# Autodesk Inventor assembly: Assembly
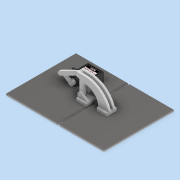
[picture p0: Inventor's stored thumbnail of the model, 180x180]
Saved by Autodesk Inventor 2020 (Build 240168000, 168)
## iProperties
Created: 2020-07-26
Part Number: Assembly
Document SubType Name: Assembly
Designer: Aarya
Author: Aarya
## Documents named in this file (10)
- C:\Users\Aarya\Downloads\R2D2_-_Servo_Driven_Hinge_Design\r2d2\Assembly.iam
- C:\Users\Aarya\Downloads\R2D2_-_Servo_Driven_Hinge_Design\r2d2\plate.ipt
- C:\Users\Aarya\Downloads\R2D2_-_Servo_Driven_Hinge_Design\r2d2\Hinge_Base.ipt
- C:\Users\Aarya\Downloads\R2D2_-_Servo_Driven_Hinge_Design\r2d2\Hinge.ipt
- C:\Users\Aarya\Downloads\R2D2_-_Servo_Driven_Hinge_Design\r2d2\horn.ipt
- C:\Users\Aarya\Downloads\R2D2_-_Servo_Driven_Hinge_Design\r2d2\horn_base.ipt
- C:\Users\Aarya\Downloads\R2D2_-_Servo_Driven_Hinge_Design\r2d2\push_rod.ipt
- C:\Users\Aarya\Downloads\R2D2_-_Servo_Driven_Hinge_Design\r2d2\SG90.ipt
- C:\Users\Aarya\Downloads\R2D2_-_Servo_Driven_Hinge_Design\r2d2\SG90 plastic Horn.ipt
- C:\Users\Aarya\Downloads\R2D2_-_Servo_Driven_Hinge_Design\r2d2\plate2.ipt
## Components (11 placed, 9 different names)
1. plate:1 — Mate:1, Mate:9
2. Hinge_Base:1 — Mate:1, Mate:2, Mate:3, Mate:4, Mate:5
3. Hinge:1 — Mate:4, Mate:5, Insert:2
4. Hinge:2 — Mate:2, Mate:3, Insert:1
5. horn:1 — Insert:1, Mate:6, Mate:7, Insert:3
6. horn:2 — Insert:2, Mate:8
7. horn_base:1 — Mate:6, Mate:7, Mate:8, Mate:10, Mate:11, Mate:12
8. push_rod:1 — Insert:3, Insert:5
9. SG90:1 — Mate:9, Angle:1, Insert:6
10. SG90 plastic Horn:1 — Insert:5, Angle:1, Insert:6
11. plate2:1 — Mate:10, Mate:11, Mate:12
## Relationships (18: Mate 12, Insert 5, Angle 1)
- Mate:1: plate:1 ↔ Hinge_Base:1
- Mate:2: Hinge_Base:1 ↔ Hinge:2
- Mate:3: Hinge_Base:1 ↔ Hinge:2
- Mate:4: Hinge_Base:1 ↔ Hinge:1
- Mate:5: Hinge_Base:1 ↔ Hinge:1
- Insert:1: Hinge:2 ↔ horn:1
- Insert:2: Hinge:1 ↔ horn:2
- Mate:6: horn:1 ↔ horn_base:1
- Mate:7: horn:1 ↔ horn_base:1
- Mate:8: horn:2 ↔ horn_base:1
- Insert:3: horn:1 ↔ push_rod:1
- Mate:9: plate:1 ↔ SG90:1
- Insert:5: push_rod:1 ↔ SG90 plastic Horn:1
- Angle:1 (60 deg): SG90:1 ↔ SG90 plastic Horn:1
- Insert:6: SG90:1 ↔ SG90 plastic Horn:1
- Mate:10: horn_base:1 ↔ plate2:1
- Mate:11: horn_base:1 ↔ plate2:1
- Mate:12: horn_base:1 ↔ plate2:1
